# Autodesk Inventor assembly: HexAndSprocketAssembly
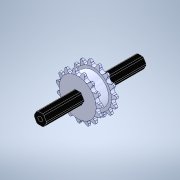
[picture p0: Inventor's stored thumbnail of the model, 180x180]
Saved by Autodesk Inventor 2021 (Build 250183000, 183)
## iProperties
Created: 2021-01-23
Part Number: HexAndSprocketAssembly
Document SubType Name: Assembly
Designer: Merkileg
Author: Merkileg
## Documents named in this file (3)
- C:\Users\Merkileg\Documents\t3-cad\HexAndSprocketAssembly.iam
- C:\Users\Merkileg\Documents\t3-cad\Archived Parts\15T Double Sprocket.ipt
- C:\Users\Merkileg\Documents\t3-cad\Archived Parts\5.5 thundershaft.ipt
## Components (2 placed, 2 different names)
1. 5.5 thundershaft:1 — Mate:1, Mate:2
2. 15T Double Sprocket:1 — Mate:1, Mate:2
## Relationships (2: Mate 2)
- Mate:1: 5.5 thundershaft:1 ↔ 15T Double Sprocket:1
- Mate:2: 5.5 thundershaft:1 ↔ 15T Double Sprocket:1
